# Autodesk Inventor assembly: hydraulic cylinder frame
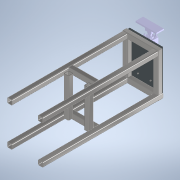
[picture p0: Inventor's stored thumbnail of the model, 180x180]
Saved by Autodesk Inventor 2022.2 (Build 262287000, 287)
## iProperties
_SolveAssemblyDoc: Frame Generator Solve Assembly
_Version: 25.0.0
Created: 2022-02-23
Part Number: hydraulic cylinder frame
Document SubType Name: Assembly
Designer: ONG
Author: ONG
## Documents named in this file (6)
- C:\Users\ONG\Documents\INVENTOR DESIGN\音箱\hydraulic cylinder frame.iam
- C:\Users\ONG\Documents\INVENTOR DESIGN\音箱\hydraulic cylinder frame line.ipt
- C:\Users\ONG\Documents\INVENTOR DESIGN\音箱\hydraulic cylinder frame\Frame\Frame 1645592768462.iam
- C:\Users\ONG\Documents\INVENTOR DESIGN\音箱\palte cylinder.ipt
- C:\Users\ONG\Downloads\hydraulic cylinder\assembly.iam
- C:\Users\ONG\Documents\INVENTOR DESIGN\音箱\hydraulic cylinder frame\Design Accelerator\Bolted Connection1.iam
## Components (5 placed, 5 different names)
1. hydraulic cylinder frame line:1
2. Frame 1645592768462:1 [sub-assembly] — Mate:1, Flush:1, Flush:2, Flush:3, Flush:4
3. palte cylinder:1 — Mate:1, Flush:1, Flush:2, Mate:2
4. assembly:1 [sub-assembly] — Mate:2, Flush:3, Flush:4, Mate:3, Mate:4
5. Bolted Connection:1 [sub-assembly] — Mate:3, Mate:4
## Relationships (8: Mate 4, Flush 4)
- Mate:1: Frame 1645592768462:1 ↔ palte cylinder:1
- Flush:1 (10 mm): Frame 1645592768462:1 ↔ palte cylinder:1
- Flush:2: Frame 1645592768462:1 ↔ palte cylinder:1
- Mate:2: palte cylinder:1 ↔ assembly:1
- Flush:3 (-70 mm): Frame 1645592768462:1 ↔ assembly:1
- Flush:4 (110 mm): Frame 1645592768462:1 ↔ assembly:1
- Mate:3: assembly:1 ↔ Bolted Connection:1
- Mate:4: assembly:1 ↔ Bolted Connection:1
